# Autodesk Inventor assembly: Assembly rupsband mirror_MIR
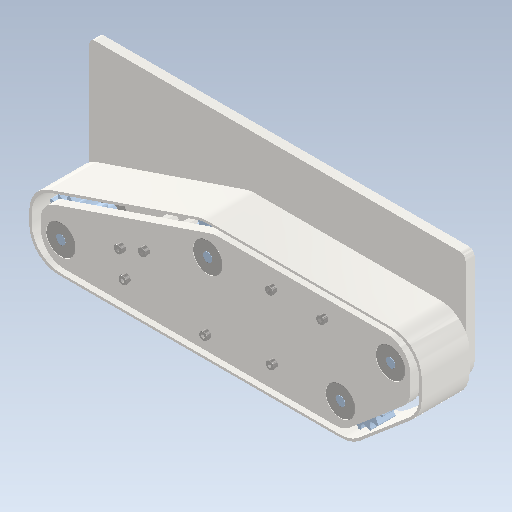
[picture p0: Inventor's stored thumbnail of the model, 512x512]
Saved by Autodesk Inventor 2021 (Build 250183000, 183)
## iProperties
Manager: PJ / DCS
Company: Emmaüs Bovenbouw Aalter
Created: 2020-11-06
Part Number: Assembly rupsband mirror_MIR
Catalog Web Link: http://emmausbovenbouw.op-weg.be/
Vendor: Emmaüs Bovenbouw Aalter
Document SubType Name: Assembly
Designer: Antho
Engineer: Declercq St.
Authority: Declercq St.
Title: Algemene Projecttitel
Author: Antho
## Documents named in this file (8)
- C:\Users\Antho\Documents\Inventor\Assembly rupsband mirror_MIR.iam
- C:\Users\Antho\Documents\Inventor\Assembly rupsband mirror_MIR.ipt
- C:\Users\Antho\Documents\Inventor\ball bearing ISO 104 - 3 73 - 8 x 26 x 8.ipt
- C:\Users\Antho\Documents\Inventor\Assembly rupsband mirror_MIR1.ipt
- C:\Users\Antho\Documents\Inventor\Assembly rupsband mirror_MIR2.ipt
- C:\Users\Antho\Documents\Inventor\Assembly rupsband mirror_MIR3.ipt
- C:\Users\Antho\Documents\Inventor\bout ISO 4762 - M4 x 16ISO.ipt
- C:\Users\Antho\Documents\Inventor\Assembly rupsband mirror_MIR4.ipt
## Components (36 placed, 3 different names)
1. Mirror Rupsband assambly:1 — Mate:1, Flush:1, Mate:4, Flush:4, Mate:3, Flush:3, Mate:2, Flush:2, Mate:6, Mate:5, Flush:5, Flush:6, Flush:7, Flush:8, Mate:22, Mate:14, Mate:20, Mate:16, Mate:18, Mate:15, Mate:21, Mate:12, Mate:19, Mate:13, Mate:17, Mate:11, Mate:39, Mate:38, Mate:37, Mate:43, Mate:41, Mate:42, Mate:40, Mate:45, Mate:44, Flush:13
2. ISO 104 (Single Direction) 3 73 - 8 x 26 x 8:1 — Mate:1, Flush:1, Mate:7
3. ISO 104 (Single Direction) 3 73 - 8 x 26 x 8:2 — Mate:4, Flush:4, Mate:10
4. ISO 104 (Single Direction) 3 73 - 8 x 26 x 8:3 — Mate:3, Flush:3, Mate:9
5. ISO 104 (Single Direction) 3 73 - 8 x 26 x 8:4 — Mate:2, Flush:2, Mate:8
6. Mirror Rupsband assambly:2 — Mate:6, Mate:5, Mate:34
7. Mirror Rupsband assambly:3 — Mate:7, Flush:5, Mate:29
8. Mirror Rupsband assambly:4 — Mate:8, Flush:6
9. Mirror Rupsband assambly:5 — Mate:9, Flush:7
10. Mirror Rupsband assambly:6 — Mate:10, Flush:8, Mate:28
11. Mirror Rupsband assambly:7 — Mate:22, Mate:14, Mate:23, Mate:32
12. Mirror Rupsband assambly:8 — Mate:20, Mate:16, Mate:30
13. Mirror Rupsband assambly:9 — Mate:18, Mate:15, Mate:35
14. Mirror Rupsband assambly:10 — Mate:21, Mate:12, Mate:33
15. Mirror Rupsband assambly:11 — Mate:19, Mate:13, Mate:31
16. Mirror Rupsband assambly:12 — Mate:17, Mate:11, Mate:36
17. Mirror Rupsband assambly:13 — Mate:23, Mate:24, Flush:9, Mate:27, Flush:10, Mate:26, Flush:11, Mate:25, Flush:12, Mate:59, Mate:52, Mate:53, Mate:47, Mate:56, Mate:49, Mate:55, Mate:46, Mate:57, Mate:50, Mate:58, Mate:51, Mate:54, Mate:48
18. ISO 104 (Single Direction) 3 73 - 8 x 26 x 8:5 — Mate:28, Mate:24, Flush:9
19. ISO 104 (Single Direction) 3 73 - 8 x 26 x 8:6 — Mate:29, Mate:27, Flush:10
20. ISO 104 (Single Direction) 3 73 - 8 x 26 x 8:7 — Mate:26, Flush:11
21. ISO 104 (Single Direction) 3 73 - 8 x 26 x 8:8 — Mate:25, Flush:12
22. ISO 4762 M4 x 16:1 — Mate:39, Mate:32
23. ISO 4762 M4 x 16:2 — Mate:38, Mate:30
24. ISO 4762 M4 x 16:3 — Mate:37, Mate:33
25. ISO 4762 M4 x 16:4 — Mate:43, Mate:36
26. ISO 4762 M4 x 16:5 — Mate:41, Mate:34
27. ISO 4762 M4 x 16:6 — Mate:42, Mate:35
28. ISO 4762 M4 x 16:7 — Mate:40, Mate:31
29. Mirror Rupsband assambly:14 — Mate:45, Mate:44, Flush:13
30. ISO 4762 M4 x 16:8 — Mate:59, Mate:52
31. ISO 4762 M4 x 16:9 — Mate:53, Mate:47
32. ISO 4762 M4 x 16:10 — Mate:56, Mate:49
33. ISO 4762 M4 x 16:11 — Mate:55, Mate:46
34. ISO 4762 M4 x 16:12 — Mate:57, Mate:50
35. ISO 4762 M4 x 16:13 — Mate:58, Mate:51
36. ISO 4762 M4 x 16:14 — Mate:54, Mate:48
## Relationships (72: Mate 59, Flush 13)
- Mate:1: Mirror Rupsband assambly:1 ↔ ISO 104 (Single Direction) 3 73 - 8 x 26 x 8:1
- Flush:1: Mirror Rupsband assambly:1 ↔ ISO 104 (Single Direction) 3 73 - 8 x 26 x 8:1
- Mate:4: Mirror Rupsband assambly:1 ↔ ISO 104 (Single Direction) 3 73 - 8 x 26 x 8:2
- Flush:4: Mirror Rupsband assambly:1 ↔ ISO 104 (Single Direction) 3 73 - 8 x 26 x 8:2
- Mate:3: Mirror Rupsband assambly:1 ↔ ISO 104 (Single Direction) 3 73 - 8 x 26 x 8:3
- Flush:3: Mirror Rupsband assambly:1 ↔ ISO 104 (Single Direction) 3 73 - 8 x 26 x 8:3
- Mate:2: Mirror Rupsband assambly:1 ↔ ISO 104 (Single Direction) 3 73 - 8 x 26 x 8:4
- Flush:2: Mirror Rupsband assambly:1 ↔ ISO 104 (Single Direction) 3 73 - 8 x 26 x 8:4
- Mate:6: Mirror Rupsband assambly:1 ↔ Mirror Rupsband assambly:2
- Mate:5: Mirror Rupsband assambly:1 ↔ Mirror Rupsband assambly:2
- Mate:7: ISO 104 (Single Direction) 3 73 - 8 x 26 x 8:1 ↔ Mirror Rupsband assambly:3
- Flush:5: Mirror Rupsband assambly:1 ↔ Mirror Rupsband assambly:3
- Mate:8: ISO 104 (Single Direction) 3 73 - 8 x 26 x 8:4 ↔ Mirror Rupsband assambly:4
- Flush:6: Mirror Rupsband assambly:1 ↔ Mirror Rupsband assambly:4
- Mate:9: ISO 104 (Single Direction) 3 73 - 8 x 26 x 8:3 ↔ Mirror Rupsband assambly:5
- Flush:7: Mirror Rupsband assambly:1 ↔ Mirror Rupsband assambly:5
- Mate:10: ISO 104 (Single Direction) 3 73 - 8 x 26 x 8:2 ↔ Mirror Rupsband assambly:6
- Flush:8: Mirror Rupsband assambly:1 ↔ Mirror Rupsband assambly:6
- Mate:22: Mirror Rupsband assambly:1 ↔ Mirror Rupsband assambly:7
- Mate:14: Mirror Rupsband assambly:1 ↔ Mirror Rupsband assambly:7
- Mate:20: Mirror Rupsband assambly:1 ↔ Mirror Rupsband assambly:8
- Mate:16: Mirror Rupsband assambly:1 ↔ Mirror Rupsband assambly:8
- Mate:18: Mirror Rupsband assambly:1 ↔ Mirror Rupsband assambly:9
- Mate:15: Mirror Rupsband assambly:1 ↔ Mirror Rupsband assambly:9
- Mate:21: Mirror Rupsband assambly:1 ↔ Mirror Rupsband assambly:10
- Mate:12: Mirror Rupsband assambly:1 ↔ Mirror Rupsband assambly:10
- Mate:19: Mirror Rupsband assambly:1 ↔ Mirror Rupsband assambly:11
- Mate:13: Mirror Rupsband assambly:1 ↔ Mirror Rupsband assambly:11
- Mate:17: Mirror Rupsband assambly:1 ↔ Mirror Rupsband assambly:12
- Mate:11: Mirror Rupsband assambly:1 ↔ Mirror Rupsband assambly:12
- Mate:23: Mirror Rupsband assambly:7 ↔ Mirror Rupsband assambly:13
- Mate:28: Mirror Rupsband assambly:6 ↔ ISO 104 (Single Direction) 3 73 - 8 x 26 x 8:5
- Mate:24: Mirror Rupsband assambly:13 ↔ ISO 104 (Single Direction) 3 73 - 8 x 26 x 8:5
- Flush:9: Mirror Rupsband assambly:13 ↔ ISO 104 (Single Direction) 3 73 - 8 x 26 x 8:5
- Mate:29: Mirror Rupsband assambly:3 ↔ ISO 104 (Single Direction) 3 73 - 8 x 26 x 8:6
- Mate:27: Mirror Rupsband assambly:13 ↔ ISO 104 (Single Direction) 3 73 - 8 x 26 x 8:6
- Flush:10: Mirror Rupsband assambly:13 ↔ ISO 104 (Single Direction) 3 73 - 8 x 26 x 8:6
- Mate:26: Mirror Rupsband assambly:13 ↔ ISO 104 (Single Direction) 3 73 - 8 x 26 x 8:7
- Flush:11: Mirror Rupsband assambly:13 ↔ ISO 104 (Single Direction) 3 73 - 8 x 26 x 8:7
- Mate:25: Mirror Rupsband assambly:13 ↔ ISO 104 (Single Direction) 3 73 - 8 x 26 x 8:8
- Flush:12: Mirror Rupsband assambly:13 ↔ ISO 104 (Single Direction) 3 73 - 8 x 26 x 8:8
- Mate:39: Mirror Rupsband assambly:1 ↔ ISO 4762 M4 x 16:1
- Mate:32: Mirror Rupsband assambly:7 ↔ ISO 4762 M4 x 16:1
- Mate:38: Mirror Rupsband assambly:1 ↔ ISO 4762 M4 x 16:2
- Mate:30: Mirror Rupsband assambly:8 ↔ ISO 4762 M4 x 16:2
- Mate:37: Mirror Rupsband assambly:1 ↔ ISO 4762 M4 x 16:3
- Mate:33: Mirror Rupsband assambly:10 ↔ ISO 4762 M4 x 16:3
- Mate:43: Mirror Rupsband assambly:1 ↔ ISO 4762 M4 x 16:4
- Mate:36: Mirror Rupsband assambly:12 ↔ ISO 4762 M4 x 16:4
- Mate:41: Mirror Rupsband assambly:1 ↔ ISO 4762 M4 x 16:5
- Mate:34: Mirror Rupsband assambly:2 ↔ ISO 4762 M4 x 16:5
- Mate:42: Mirror Rupsband assambly:1 ↔ ISO 4762 M4 x 16:6
- Mate:35: Mirror Rupsband assambly:9 ↔ ISO 4762 M4 x 16:6
- Mate:40: Mirror Rupsband assambly:1 ↔ ISO 4762 M4 x 16:7
- Mate:31: Mirror Rupsband assambly:11 ↔ ISO 4762 M4 x 16:7
- Mate:45 (8 mm): Mirror Rupsband assambly:1 ↔ Mirror Rupsband assambly:14
- Mate:44 (5 mm): Mirror Rupsband assambly:1 ↔ Mirror Rupsband assambly:14
- Flush:13: Mirror Rupsband assambly:1 ↔ Mirror Rupsband assambly:14
- Mate:59: Mirror Rupsband assambly:13 ↔ ISO 4762 M4 x 16:8
- Mate:52: Mirror Rupsband assambly:13 ↔ ISO 4762 M4 x 16:8
- Mate:53: Mirror Rupsband assambly:13 ↔ ISO 4762 M4 x 16:9
- Mate:47: Mirror Rupsband assambly:13 ↔ ISO 4762 M4 x 16:9
- Mate:56: Mirror Rupsband assambly:13 ↔ ISO 4762 M4 x 16:10
- Mate:49: Mirror Rupsband assambly:13 ↔ ISO 4762 M4 x 16:10
- Mate:55: Mirror Rupsband assambly:13 ↔ ISO 4762 M4 x 16:11
- Mate:46: Mirror Rupsband assambly:13 ↔ ISO 4762 M4 x 16:11
- Mate:57: Mirror Rupsband assambly:13 ↔ ISO 4762 M4 x 16:12
- Mate:50: Mirror Rupsband assambly:13 ↔ ISO 4762 M4 x 16:12
- Mate:58: Mirror Rupsband assambly:13 ↔ ISO 4762 M4 x 16:13
- Mate:51: Mirror Rupsband assambly:13 ↔ ISO 4762 M4 x 16:13
- Mate:54: Mirror Rupsband assambly:13 ↔ ISO 4762 M4 x 16:14
- Mate:48: Mirror Rupsband assambly:13 ↔ ISO 4762 M4 x 16:14
